# Autodesk Inventor assembly: obj3
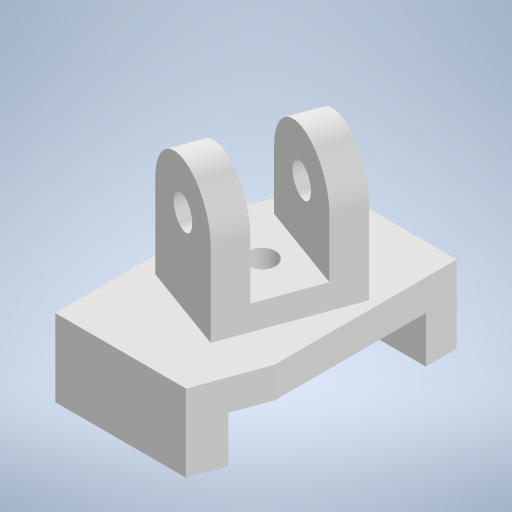
[picture p0: Inventor's stored thumbnail of the model, 512x512]
Saved by Autodesk Inventor 2023.2 (Build 272271030, 271C)
## iProperties
Created: 2023-02-25
Part Number: obj3
Document SubType Name: Assembly
Designer: Cris Pat
Author: Cris Pat
## Documents named in this file (5)
- C:\Users\Cris Pat\Desktop\U\Semestre 9\disenio e innovacion\CAD\obj3.iam
- C:\Users\Cris Pat\Desktop\U\Semestre 9\disenio e innovacion\CAD\base_obj3.ipt
- C:\Users\Cris Pat\Desktop\U\Semestre 9\disenio e innovacion\CAD\cuerpo_obj3.ipt
- C:\Users\Cris Pat\Documents\Inventor\Content Center Files\R2023\en-US\DIN 439-2\DIN 439 - M5 x 0.8.ipt
- C:\Users\Cris Pat\Documents\Inventor\Content Center Files\R2023\en-US\DIN 84\DIN 84 - M5 x 10.ipt
## Components (4 placed, 4 different names)
1. base_obj3:1 — Rigid:1, Rotational:2
2. cuerpo_obj3:1 — Rigid:1, Rotational:1
3. DIN 439-2 - replaced by DIN EN 24035/28675 M5:1 — Rotational:2
4. DIN 84 - replaced by DIN EN ISO 1207 M5 x 10:1 — Rotational:1
## Relationships (3: RevoluteJoint 2, WeldJoint 1)
- Rigid:1 [WeldJoint]: base_obj3:1 ↔ cuerpo_obj3:1
- Rotational:1 [RevoluteJoint]: cuerpo_obj3:1 ↔ DIN 84 - replaced by DIN EN ISO 1207 M5 x 10:1
- Rotational:2 [RevoluteJoint]: base_obj3:1 ↔ DIN 439-2 - replaced by DIN EN 24035/28675 M5:1
